# Autodesk Inventor assembly: Wades extruder
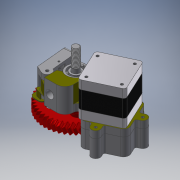
[picture p0: Inventor's stored thumbnail of the model, 180x180]
Saved by Autodesk Inventor 2016 SP1 (Build 200210100, 210)
## iProperties
Created: 2015-11-17
Part Number: Wades extruder
Document SubType Name: Assembly
Designer: PowerStation9000
Author: PowerStation9000
## Documents named in this file (9)
- C:\Users\PowerStation9000\AppData\Local\Autodesk\Autodesk Sync\Cloud\mathiaslk\UltiBot mk2\Min Wades Extruder\Ultibot v2\Wades extruder.iam
- C:\Users\PowerStation9000\AppData\Local\Autodesk\Autodesk Sync\Cloud\mathiaslk\UltiBot mk2\Min Wades Extruder\Engranaje1_Grande_47.ipt
- C:\Users\PowerStation9000\AppData\Local\Autodesk\Autodesk Sync\Cloud\mathiaslk\UltiBot mk2\Min Wades Extruder\Engranaje2_Pequeo_9.ipt
- C:\Users\PowerStation9000\AppData\Local\Autodesk\Autodesk Sync\Cloud\mathiaslk\UltiBot mk2\Min Wades Extruder\Wades 17m2.ipt
- C:\Users\PowerStation9000\AppData\Local\Autodesk\Autodesk Sync\Cloud\mathiaslk\UltiBot mk2\Importerede komponenter\NEMA 17 stepper motor\40mm\Nema17 - 40mm BRUG DENNE.ipt
- C:\Users\PowerStation9000\AppData\Local\Autodesk\Autodesk Sync\Cloud\mathiaslk\UltiBot mk2\Min Wades Extruder\Filament holder.ipt
- C:\Users\PowerStation9000\AppData\Local\Autodesk\Autodesk Sync\Cloud\mathiaslk\UltiBot mk2\Min Wades Extruder\Hobbled Bolt.ipt
- C:\Users\PowerStation9000\AppData\Local\Autodesk\Autodesk Sync\Cloud\mathiaslk\UltiBot mk2\Min Wades Extruder\8mm Bearing SKF 608 RS 286-7530 v1.ipt
- C:\Users\PowerStation9000\AppData\Local\Autodesk\Autodesk Sync\Cloud\mathiaslk\UltiBot mk2\Min Wades Extruder\Adapter.ipt
## Components (10 placed, 8 different names)
1. Engranaje1_Grande_47:1 — Mate:1, Mate:2, Flush:1, Rotation:1, Mate:13, Angle:1, Mate:14
2. Engranaje2_Pequeo_9:1 — Mate:6, Flush:1, Rotation:1
3. Wades 17m2:1 — Mate:1, Mate:2, Mate:3, Mate:4, Mate:7, Flush:2, Mate:8, Flush:3, Mate:11, Mate:12, Angle:2, Flush:4
4. Nema17 - 40mm BRUG DENNE:1 — Mate:3, Mate:4, Mate:6, Angle:2
5. Filament holder:1 — Mate:9, Mate:10, Mate:11, Mate:12
6. Hobbled Bolt:1 — Mate:13, Angle:1, Mate:14
7. 8mm Bearing SKF 608 RS 286-7530 v1:1 — Mate:8, Flush:3
8. 8mm Bearing SKF 608 RS 286-7530 v1:2 — Mate:7, Flush:2
9. 8mm Bearing SKF 608 RS 286-7530 v1:3 — Mate:9, Mate:10
10. Adapter:1 — Flush:4
## Relationships (20: Mate 13, Flush 4, Angle 2, RelateRotation 1)
- Mate:1: Engranaje1_Grande_47:1 ↔ Wades 17m2:1
- Mate:2 (1 mm): Engranaje1_Grande_47:1 ↔ Wades 17m2:1
- Mate:3: Wades 17m2:1 ↔ Nema17 - 40mm BRUG DENNE:1
- Mate:4: Wades 17m2:1 ↔ Nema17 - 40mm BRUG DENNE:1
- Mate:6: Engranaje2_Pequeo_9:1 ↔ Nema17 - 40mm BRUG DENNE:1
- Flush:1: Engranaje1_Grande_47:1 ↔ Engranaje2_Pequeo_9:1
- Rotation:1 [RelateRotation] (5.2222 ul): Engranaje1_Grande_47:1 ↔ Engranaje2_Pequeo_9:1
- Mate:7: Wades 17m2:1 ↔ 8mm Bearing SKF 608 RS 286-7530 v1:2
- Flush:2: Wades 17m2:1 ↔ 8mm Bearing SKF 608 RS 286-7530 v1:2
- Mate:8: Wades 17m2:1 ↔ 8mm Bearing SKF 608 RS 286-7530 v1:1
- Flush:3 (-1 mm): Wades 17m2:1 ↔ 8mm Bearing SKF 608 RS 286-7530 v1:1
- Mate:9: Filament holder:1 ↔ 8mm Bearing SKF 608 RS 286-7530 v1:3
- Mate:10: Filament holder:1 ↔ 8mm Bearing SKF 608 RS 286-7530 v1:3
- Mate:11: Wades 17m2:1 ↔ Filament holder:1
- Mate:12: Wades 17m2:1 ↔ Filament holder:1
- Mate:13: Engranaje1_Grande_47:1 ↔ Hobbled Bolt:1
- Angle:1 (0 deg): Engranaje1_Grande_47:1 ↔ Hobbled Bolt:1
- Mate:14: Engranaje1_Grande_47:1 ↔ Hobbled Bolt:1
- Angle:2 (0 deg): Wades 17m2:1 ↔ Nema17 - 40mm BRUG DENNE:1
- Flush:4: Wades 17m2:1 ↔ Adapter:1
